# Autodesk Inventor assembly: crankshaft assembly
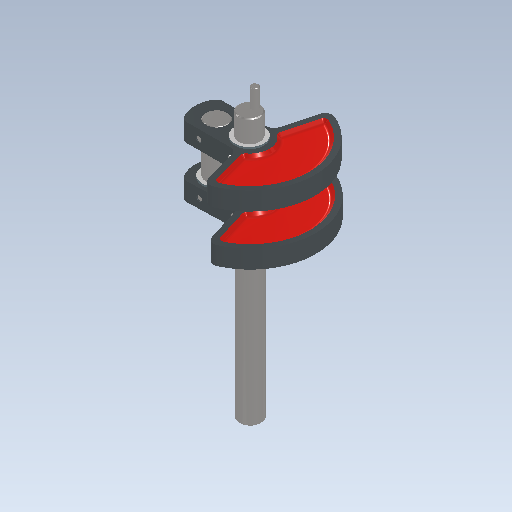
[picture p0: Inventor's stored thumbnail of the model, 512x512]
Saved by Autodesk Inventor 2020 (Build 240168000, 168)
## iProperties
Created: 2020-08-08
Part Number: crankshaft assembly
Document SubType Name: Assembly
Designer: benny
Author: benny
## Documents named in this file (6)
- C:\Users\benny\Desktop\importantmajorprojecthev_june\engine\crankshaft assembly\BENNY S L_JUNE BATCH_crankshaft assembly.iam
- C:\Users\benny\Desktop\importantmajorprojecthev_june\engine\crankshaft assembly\BENNY S L_JUNE BATCH_crankshaft counter weight.ipt
- C:\Users\benny\Desktop\importantmajorprojecthev_june\engine\crankshaft assembly\BENNY S L_JUNE BATCH_crankshaft pin.ipt
- C:\Users\benny\Desktop\importantmajorprojecthev_june\engine\crankshaft assembly\BENNY S L_JUNE BATCH_crankshaft valve crank.ipt
- C:\Users\benny\Desktop\importantmajorprojecthev_june\engine\crankshaft assembly\BENNY S L_JUNE BATCH_crankshaft.ipt
- C:\Users\benny\Documents\Inventor\Content Center Files\R2020\en-US\ISO 2338(2)\ISO 2338 - 3 h8 x 20.ipt
## Components (9 placed, 5 different names)
1. BENNY S L_JUNE BATCH_crankshaft counter weight:1 — Mate:8, Mate:9, Mate:13, Mate:14, Insert:3, Insert:4
2. BENNY S L_JUNE BATCH_crankshaft counter weight:2 — Mate:6, Mate:7, Mate:15, Mate:16, Insert:1, Insert:2
3. BENNY S L_JUNE BATCH_crankshaft valve crank:1 — Mate:6, Mate:7
4. BENNY S L_JUNE BATCH_crankshaft:1 — Mate:8, Mate:9
5. BENNY S L_JUNE BATCH_crankshaft pin:2 — Mate:13, Mate:14, Mate:15, Mate:16
6. ISO 2338 3 h8 x 20:1 — Insert:1
7. ISO 2338 3 h8 x 20:2 — Insert:2
8. ISO 2338 3 h8 x 20:3 — Insert:4
9. ISO 2338 3 h8 x 20:4 — Insert:3
## Relationships (12: Mate 8, Insert 4)
- Mate:6: BENNY S L_JUNE BATCH_crankshaft counter weight:2 ↔ BENNY S L_JUNE BATCH_crankshaft valve crank:1
- Mate:7: BENNY S L_JUNE BATCH_crankshaft counter weight:2 ↔ BENNY S L_JUNE BATCH_crankshaft valve crank:1
- Mate:8: BENNY S L_JUNE BATCH_crankshaft counter weight:1 ↔ BENNY S L_JUNE BATCH_crankshaft:1
- Mate:9: BENNY S L_JUNE BATCH_crankshaft counter weight:1 ↔ BENNY S L_JUNE BATCH_crankshaft:1
- Mate:13: BENNY S L_JUNE BATCH_crankshaft counter weight:1 ↔ BENNY S L_JUNE BATCH_crankshaft pin:2
- Mate:14: BENNY S L_JUNE BATCH_crankshaft counter weight:1 ↔ BENNY S L_JUNE BATCH_crankshaft pin:2
- Mate:15: BENNY S L_JUNE BATCH_crankshaft counter weight:2 ↔ BENNY S L_JUNE BATCH_crankshaft pin:2
- Mate:16: BENNY S L_JUNE BATCH_crankshaft counter weight:2 ↔ BENNY S L_JUNE BATCH_crankshaft pin:2
- Insert:1: BENNY S L_JUNE BATCH_crankshaft counter weight:2 ↔ ISO 2338 3 h8 x 20:1
- Insert:2: BENNY S L_JUNE BATCH_crankshaft counter weight:2 ↔ ISO 2338 3 h8 x 20:2
- Insert:3: BENNY S L_JUNE BATCH_crankshaft counter weight:1 ↔ ISO 2338 3 h8 x 20:4
- Insert:4: BENNY S L_JUNE BATCH_crankshaft counter weight:1 ↔ ISO 2338 3 h8 x 20:3
